# Autodesk Inventor assembly: HbMRLFinger
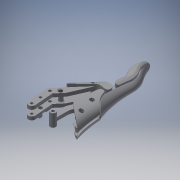
[picture p0: Inventor's stored thumbnail of the model, 180x180]
Saved by Autodesk Inventor 2018 (Build 220112000, 112)
## iProperties
Part Number: HbMRLFinger
Material: 一般
Document SubType Name: Assembly
Designer: sktom
Author: sktom
## Documents named in this file (8)
- D:\OneDrive\CAD\MAJ\hackberry\HACKberry-hardware\3D_69%inlength\Inventor\HbHandForChild\HbFinger01ForChild\HbFinger01ForChild.iam
- D:\OneDrive\CAD\MAJ\hackberry\HACKberry-hardware\3D_69%inlength\Inventor\HbHandForChild\HbFinger01ForChild\HbCouplerLinkCover03ForChild.ipt
- D:\OneDrive\CAD\MAJ\hackberry\HACKberry-hardware\3D_69%inlength\Inventor\HbHandForChild\HbFinger01ForChild\HbCouplerLink02ForChild.ipt
- D:\OneDrive\CAD\MAJ\hackberry\HACKberry-hardware\3D_69%inlength\Inventor\HbHandForChild\HbFinger01ForChild\HbMiddle-DistalPhalanx02ForChild.ipt
- D:\OneDrive\CAD\MAJ\hackberry\HACKberry-hardware\3D_69%inlength\Inventor\HbHandForChild\HbFinger01ForChild\HbProximalPhalanx02ForChild.ipt
- D:\OneDrive\CAD\MAJ\hackberry\HACKberry-hardware\3D_69%inlength\Inventor\HbHandForChild\HbFinger01ForChild\HbProximalPhalanxCover02ForChild.ipt
- D:\OneDrive\CAD\MAJ\hackberry\HACKberry-hardware\3D_69%inlength\Inventor\HbHandForChild\HbFinger01ForChild\shaft_phi1.5_l6.ipt
- D:\OneDrive\CAD\MAJ\hackberry\HACKberry-hardware\3D_69%inlength\Inventor\HbHandForChild\HbFinger01ForChild\bolt_M1.4L6.ipt
## Components (11 placed, 7 different names)
1. HbCouplerLinkCover03ForChild:1 — 挿入:7, 挿入:8, 挿入:9
2. HbCouplerLink02ForChild:1 — 挿入:8, 挿入:9, 挿入:11, 挿入:12
3. HbMiddle-DistalPhalanx02ForChild:1 — リジッド:1, リジッド:2, 挿入:7, 挿入:10
4. HbProximalPhalanx02ForChild:1 — 挿入:5, 挿入:6
5. HbProximalPhalanxCover02ForChild:1 — 挿入:5, 挿入:6, 挿入:10, 挿入:13, 挿入:14
6. shaft_phi1.5_l6:1 — リジッド:1
7. shaft_phi1.5_l6:2 — リジッド:2
8. bolt_M1.4L6:1 — 挿入:11
9. bolt_M1.4L6:2 — 挿入:12
10. bolt_M1.4L6:3 — 挿入:13
11. bolt_M1.4L6:4 — 挿入:14
## Relationships (12: Insert 10, WeldJoint 2)
- 挿入:5 [Insert]: HbProximalPhalanx02ForChild:1 ↔ HbProximalPhalanxCover02ForChild:1
- 挿入:6 [Insert]: HbProximalPhalanx02ForChild:1 ↔ HbProximalPhalanxCover02ForChild:1
- リジッド:1 [WeldJoint]: HbMiddle-DistalPhalanx02ForChild:1 ↔ shaft_phi1.5_l6:1
- リジッド:2 [WeldJoint]: HbMiddle-DistalPhalanx02ForChild:1 ↔ shaft_phi1.5_l6:2
- 挿入:7 [Insert] (0.05 mm): HbCouplerLinkCover03ForChild:1 ↔ HbMiddle-DistalPhalanx02ForChild:1
- 挿入:8 [Insert]: HbCouplerLinkCover03ForChild:1 ↔ HbCouplerLink02ForChild:1
- 挿入:9 [Insert]: HbCouplerLinkCover03ForChild:1 ↔ HbCouplerLink02ForChild:1
- 挿入:10 [Insert] (0.1 mm): HbMiddle-DistalPhalanx02ForChild:1 ↔ HbProximalPhalanxCover02ForChild:1
- 挿入:11 [Insert]: HbCouplerLink02ForChild:1 ↔ bolt_M1.4L6:1
- 挿入:12 [Insert]: HbCouplerLink02ForChild:1 ↔ bolt_M1.4L6:2
- 挿入:13 [Insert]: HbProximalPhalanxCover02ForChild:1 ↔ bolt_M1.4L6:3
- 挿入:14 [Insert]: HbProximalPhalanxCover02ForChild:1 ↔ bolt_M1.4L6:4
